# Autodesk Inventor assembly: Assy_arm
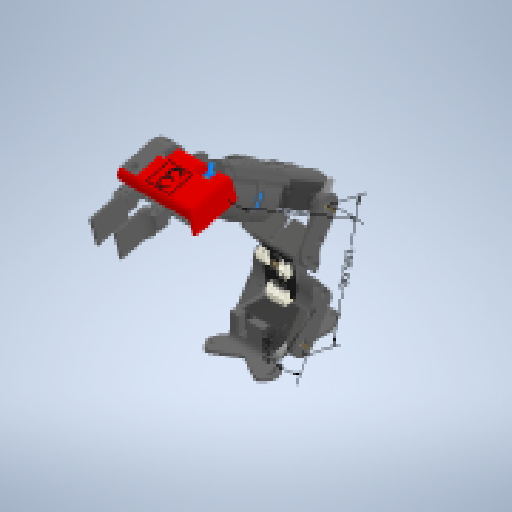
[picture p0: Inventor's stored thumbnail of the model, 512x512]
Saved by Autodesk Inventor 2024.1 (Build 281209000, 209)
## iProperties
Created: 2025-03-03
Part Number: Assy_arm
Document SubType Name: Assembly
Designer: hibik
Author: hibik
## Documents named in this file (5)
- C:\Users\hibik\Documents\Robomech\RESCUE\ORCA\hard\arm\Assy_arm.iam
- C:\Users\hibik\Documents\Robomech\RESCUE\ORCA\hard\arm\Assy_wrist.iam
- C:\Users\hibik\Documents\Robomech\RESCUE\ORCA\hard\arm\Assy_hand.iam
- C:\Users\hibik\Documents\Robomech\RESCUE\ORCA\hard\arm\Assy_fore_arm.iam
- C:\Users\hibik\Documents\Robomech\RESCUE\ORCA\hard\arm\Assy_upper_arm.iam
## Components (4 placed, 4 different names)
1. Assy_fore_arm:1 [sub-assembly] — 挿入:3, 挿入:4
2. Assy_hand:1 [sub-assembly] — 挿入:5
3. Assy_wrist:1 [sub-assembly] — 挿入:4, 挿入:5
4. Assy_upper_arm:1 [sub-assembly] — 挿入:3
## Relationships (3: Insert 3)
- 挿入:3 [Insert]: Assy_fore_arm:1 ↔ Assy_upper_arm:1
- 挿入:4 [Insert]: Assy_fore_arm:1 ↔ Assy_wrist:1
- 挿入:5 [Insert]: Assy_hand:1 ↔ Assy_wrist:1
